# Autodesk Inventor assembly: HPC+LPC
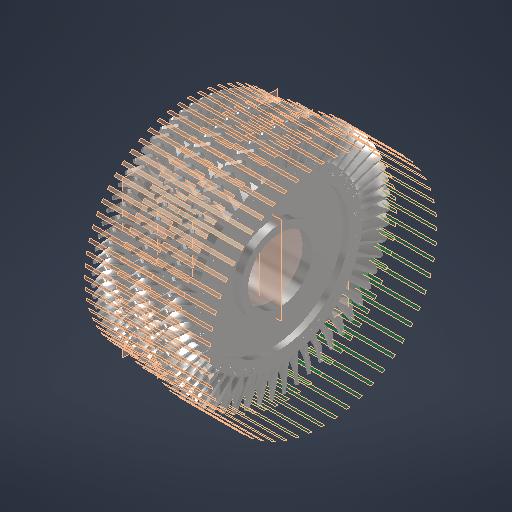
[picture p0: Inventor's stored thumbnail of the model, 512x512]
Saved by Autodesk Inventor 2026.2 (Build 302298010, 298A)
## iProperties
Created: 2026-04-26
Part Number: HPC+LPC
Document SubType Name: Assembly
Designer: Yan
Author: Yan
## Documents named in this file (5)
- C:\Users\Yan\Desktop\Turbina\HPC+LPC.iam
- C:\Users\Yan\Desktop\Turbina\Stadio9.iam
- C:\Users\Yan\Desktop\Turbina\Stadio10.iam
- C:\Users\Yan\Desktop\Turbina\Stadio8.iam
- C:\Users\Yan\Desktop\Turbina\Spaziamento8-9-10ipt.ipt
## Components (5 placed, 4 different names)
1. Stadio9:1 [sub-assembly] — Mate:3, Mate:4, Mate:5, Mate:6
2. Stadio10:1 [sub-assembly] — Mate:1, Mate:2, Mate:4, Mate:8
3. Stadio8:1 [sub-assembly] — Mate:7, Mate:8
4. Spaziamento8-9-10ipt:1 — Mate:1, Mate:2, Mate:3
5. Spaziamento8-9-10ipt:2 — Mate:5, Mate:6, Mate:7
## Relationships (8: Mate 8)
- Mate:1: Stadio10:1 ↔ Spaziamento8-9-10ipt:1
- Mate:2: Stadio10:1 ↔ Spaziamento8-9-10ipt:1
- Mate:3: Stadio9:1 ↔ Spaziamento8-9-10ipt:1
- Mate:4: Stadio9:1 ↔ Stadio10:1
- Mate:5: Stadio9:1 ↔ Spaziamento8-9-10ipt:2
- Mate:6: Stadio9:1 ↔ Spaziamento8-9-10ipt:2
- Mate:7: Stadio8:1 ↔ Spaziamento8-9-10ipt:2
- Mate:8: Stadio10:1 ↔ Stadio8:1
